# Autodesk Inventor assembly: derive_rod_v7
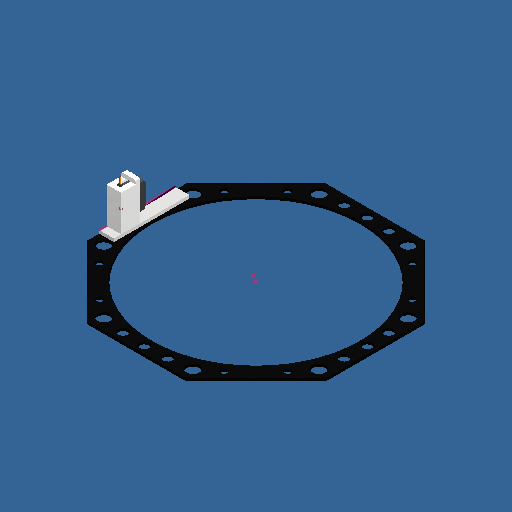
[picture p0: Inventor's stored thumbnail of the model, 512x512]
Saved by Autodesk Inventor 2026.2 (Build 302298000, 298)
## iProperties
Created: 2026-01-13
Part Number: derive_rod_v7
Document SubType Name: Assembly
Designer: Thoma
Author: Thoma
## Documents named in this file (6)
- C:\Users\Thoma\OneDrive\Desktop\dir\telescope_cover\cover\derive_casing.iam
- C:\Users\Thoma\OneDrive\Desktop\dir\telescope_cover\telescope\version_3\Telescope_End.ipt
- C:\Users\Thoma\OneDrive\Desktop\dir\telescope_cover\cover\Cover_Upper_v3.ipt
- C:\Users\Thoma\OneDrive\Desktop\dir\telescope_cover\cover\Base_Plate_v2.ipt
- C:\Users\Thoma\OneDrive\Desktop\dir\telescope_cover\servo\DSS-M15S Servo.ipt
- C:\Users\Thoma\OneDrive\Desktop\dir\telescope_cover\cover\casing_v2.ipt
## Components (5 placed, 5 different names)
1. Telescope_End:1 — Mate:3, Mate:4, Mate:5, Flush:1
2. Cover_Upper_v3:1
3. Base_Plate_v2:1 — Mate:3, Mate:4, Mate:5, Mate:6, Flush:8
4. DSS-M15S Servo:1 — Mate:6, Flush:1, Flush:8, Mate:12, Mate:13, Mate:14
5. casing_v2:1 — Mate:12, Mate:13, Mate:14
## Relationships (9: Mate 7, Flush 2)
- Mate:3: Telescope_End:1 ↔ Base_Plate_v2:1
- Mate:4: Telescope_End:1 ↔ Base_Plate_v2:1
- Mate:5: Telescope_End:1 ↔ Base_Plate_v2:1
- Mate:6 (14 mm): Base_Plate_v2:1 ↔ DSS-M15S Servo:1
- Flush:1 (2.5 mm): Telescope_End:1 ↔ DSS-M15S Servo:1
- Flush:8 (13.475 mm): Base_Plate_v2:1 ↔ DSS-M15S Servo:1
- Mate:12: DSS-M15S Servo:1 ↔ casing_v2:1
- Mate:13 (1.1 mm): DSS-M15S Servo:1 ↔ casing_v2:1
- Mate:14 (0.1 mm): DSS-M15S Servo:1 ↔ casing_v2:1
